# Autodesk Inventor assembly: Diaphragm
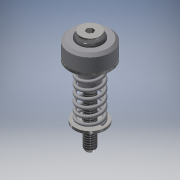
[picture p0: Inventor's stored thumbnail of the model, 180x180]
Saved by Autodesk Inventor 2018 (Build 220112000, 112)
## iProperties
Created: 2020-03-27
Part Number: Diaphragm
Document SubType Name: Assembly
Designer: emile
Author: emile
## Documents named in this file (8)
- C:\Users\emile\OneDrive\Documents\Inventor\Respirator\Peep\Diaphragm.iam
- C:\Users\emile\OneDrive\Documents\Inventor\Respirator\Peep\Diaphragme.ipt
- C:\Users\emile\OneDrive\Documents\Inventor\Respirator\Peep\High-Temperature Silicone O-Ring(1283N198).ipt
- C:\Users\emile\OneDrive\Documents\Inventor\Content Center Files\R2018\en-US\ANSI B18.22.1\ANSI B18.22.1 - 1_4 - wide - Type B.ipt
- C:\Users\emile\OneDrive\Documents\Inventor\Respirator\Peep\9435K137_302 SS CORROSION-RST  SPRINGS.ipt
- C:\Users\emile\OneDrive\Documents\Inventor\Respirator\Peep\alignspring.ipt
- C:\Users\emile\OneDrive\Documents\Inventor\Content Center Files\R2018\en-US\ANSI B18.3(04)\ANSI B18.3 - 1_4-20 UNC - 2.5(30).ipt
- C:\Users\emile\OneDrive\Documents\Inventor\Content Center Files\R2018\en-US\ANSI B18.22.1\ANSI B18.22.1 - 1_4 - Regular - Type B.ipt
## Components (7 placed, 7 different names)
1. Diaphragme:1 — Flush:1, Flush:2, Mate:3, Mate:6, Mate:10, Tangent:4, Mate:12
2. High-Temperature Silicone O-Ring(1283N198):1 — Mate:10, Tangent:4, Tangent:5
3. Hexagon Socket Flat Countersunk Head Cap Screw - Inch 1/4-20 UNC x 2.5:1 — Mate:12, Tangent:5, Mate:14, Mate:16, Mate:18
4. Plain Washer (Inch) 1/4 - wide - Type B:1 — Mate:6, Mate:15, Mate:17
5. 9435K137_302 SS CORROSION-RST  SPRINGS:1 — Mate:15, Mate:16, Mate:19
6. alignspring:1 — Mate:14, Mate:17
7. Plain Washer (Inch) 1/4 - Regular - Type B:1 — Mate:18, Mate:19
## Relationships (14: Mate 10, Flush 2, Tangent 2)
- Flush:1: Diaphragme:1
- Flush:2: Diaphragme:1
- Mate:3: Diaphragme:1
- Mate:6: Diaphragme:1 ↔ Plain Washer (Inch) 1/4 - wide - Type B:1
- Mate:10: Diaphragme:1 ↔ High-Temperature Silicone O-Ring(1283N198):1
- Tangent:4: Diaphragme:1 ↔ High-Temperature Silicone O-Ring(1283N198):1
- Mate:12: Diaphragme:1 ↔ Hexagon Socket Flat Countersunk Head Cap Screw - Inch 1/4-20 UNC x 2.5:1
- Tangent:5: High-Temperature Silicone O-Ring(1283N198):1 ↔ Hexagon Socket Flat Countersunk Head Cap Screw - Inch 1/4-20 UNC x 2.5:1
- Mate:14: Hexagon Socket Flat Countersunk Head Cap Screw - Inch 1/4-20 UNC x 2.5:1 ↔ alignspring:1
- Mate:15: Plain Washer (Inch) 1/4 - wide - Type B:1 ↔ 9435K137_302 SS CORROSION-RST  SPRINGS:1
- Mate:16: Hexagon Socket Flat Countersunk Head Cap Screw - Inch 1/4-20 UNC x 2.5:1 ↔ 9435K137_302 SS CORROSION-RST  SPRINGS:1
- Mate:17: Plain Washer (Inch) 1/4 - wide - Type B:1 ↔ alignspring:1
- Mate:18: Hexagon Socket Flat Countersunk Head Cap Screw - Inch 1/4-20 UNC x 2.5:1 ↔ Plain Washer (Inch) 1/4 - Regular - Type B:1
- Mate:19: 9435K137_302 SS CORROSION-RST  SPRINGS:1 ↔ Plain Washer (Inch) 1/4 - Regular - Type B:1
